# Autodesk Inventor assembly: Steam Engine 2 inch
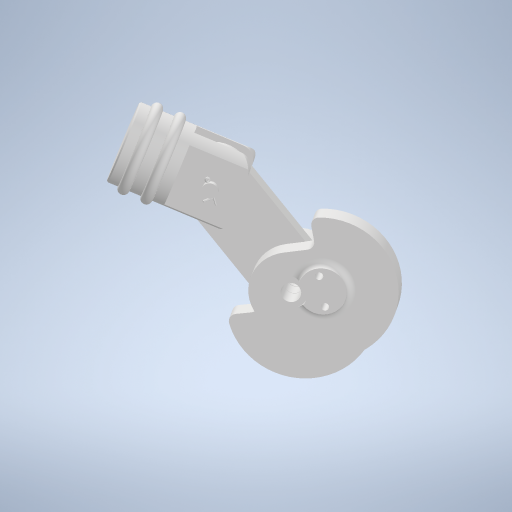
[picture p0: Inventor's stored thumbnail of the model, 512x512]
Saved by Autodesk Inventor 2023 (Build 270158000, 158)
## iProperties
Created: 2022-10-29
Part Number: Steam Engine 2 inch
Document SubType Name: Assembly
Designer: tommy
Author: tommy
## Documents named in this file (9)
- C:\Users\tommy\Documents\Repositories\Steam Engine\2 inch Design V2\Steam Engine 2 inch V2.iam
- C:\Users\tommy\Documents\Repositories\Steam Engine\2 inch Design V2\Wrist Pin Bearing.ipt
- C:\Users\tommy\Documents\Repositories\Steam Engine\2 inch Design V2\Piston O Ring.ipt
- C:\Users\tommy\Documents\Repositories\Steam Engine\2 inch Design V2\Piston Head.ipt
- C:\Users\tommy\Documents\Repositories\Steam Engine\2 inch Design V2\Crank on Crankshaft 2.ipt
- C:\Users\tommy\Documents\Repositories\Steam Engine\2 inch Design V2\Connecting Rod.ipt
- C:\Users\tommy\Documents\Repositories\Steam Engine\2 inch Design V2\Connecting Rod Bearing.ipt
- C:\Users\tommy\Documents\Repositories\Steam Engine\2 inch Design V2\Wrist Pin.ipt
- C:\Users\tommy\Documents\Repositories\Steam Engine\2 inch Design V2\Cotter Pin.ipt
## Components (11 placed, 8 different names)
1. Crank on Crankshaft 2:1 — Mate:8, Mate:9
2. Crank on Crankshaft 2:2 — Mate:5, Mate:7
3. Piston Head:1 — Mate:1, Mate:2, Mate:3, Tangent:1, Tangent:2, Mate:10, Mate:11, Mate:14, Mate:16
4. Connecting Rod:1 — Mate:4, Flush:1, Mate:6, Flush:2, Mate:7, Mate:8, Mate:15, Mate:16
5. Piston O Ring:1 — Mate:3, Tangent:1
6. Piston O Ring:2 — Mate:2, Tangent:2
7. Wrist Pin Bearing:1 — Mate:1, Mate:4, Flush:1, Mate:10, Mate:15
8. Connecting Rod Bearing:1 — Mate:5, Mate:6, Flush:2, Mate:9
9. Wrist Pin:1 — Mate:11, Mate:12, Tangent:4, Mate:13, Tangent:5
10. Cotter Pin:2 — Mate:12, Tangent:4, Mate:14, Angle:1
11. Cotter Pin:3 — Mate:13, Tangent:5, Angle:1
## Relationships (23: Mate 16, Tangent 4, Flush 2, Angle 1)
- Mate:1: Piston Head:1 ↔ Wrist Pin Bearing:1
- Mate:2: Piston Head:1 ↔ Piston O Ring:2
- Mate:3: Piston Head:1 ↔ Piston O Ring:1
- Tangent:1: Piston Head:1 ↔ Piston O Ring:1
- Tangent:2: Piston Head:1 ↔ Piston O Ring:2
- Mate:4: Connecting Rod:1 ↔ Wrist Pin Bearing:1
- Flush:1: Connecting Rod:1 ↔ Wrist Pin Bearing:1
- Mate:5: Crank on Crankshaft 2:2 ↔ Connecting Rod Bearing:1
- Mate:6: Connecting Rod:1 ↔ Connecting Rod Bearing:1
- Flush:2: Connecting Rod:1 ↔ Connecting Rod Bearing:1
- Mate:7: Crank on Crankshaft 2:2 ↔ Connecting Rod:1
- Mate:8: Crank on Crankshaft 2:1 ↔ Connecting Rod:1
- Mate:9: Crank on Crankshaft 2:1 ↔ Connecting Rod Bearing:1
- Mate:10: Piston Head:1 ↔ Wrist Pin Bearing:1
- Mate:11: Piston Head:1 ↔ Wrist Pin:1
- Mate:12: Wrist Pin:1 ↔ Cotter Pin:2
- Tangent:4: Wrist Pin:1 ↔ Cotter Pin:2
- Mate:13: Wrist Pin:1 ↔ Cotter Pin:3
- Tangent:5: Wrist Pin:1 ↔ Cotter Pin:3
- Mate:14: Piston Head:1 ↔ Cotter Pin:2
- Angle:1 (0 deg): Cotter Pin:2 ↔ Cotter Pin:3
- Mate:15: Connecting Rod:1 ↔ Wrist Pin Bearing:1
- Mate:16: Piston Head:1 ↔ Connecting Rod:1
